# Autodesk Inventor assembly: Tattu 850mah 4S
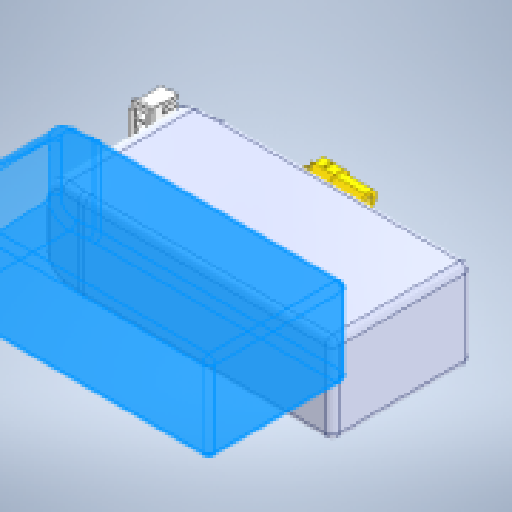
[picture p0: Inventor's stored thumbnail of the model, 512x512]
Saved by Autodesk Inventor 2023.2 (Build 272271000, 271)
## iProperties
Created: 2022-12-23
Part Number: Tattu 850mah 4S
Document SubType Name: Assembly
Designer: Nathan Cai
Mass: 57 g
Surface Area: 117.721 cm^2
Volume: 1.48579 cm^3
Density: 43.3194 g/cm^3
Author: Nathan Cai
## Documents named in this file (4)
- C:\Users\Nathan Cai\Documents\Inventor\Moon Cake V0.15\Tattu 4S 850mah\Tattu 850mah 4S.iam
- C:\Users\Nathan Cai\Documents\Inventor\Moon Cake V0.15\Tattu 4S 850mah\FUNDA 13.ipt
- C:\Users\Nathan Cai\Documents\Inventor\Moon Cake V0.15\Tattu 4S 850mah\JST XHP-4.ipt
- C:\Users\Nathan Cai\Documents\Inventor\Moon Cake V0.15\Tattu 4S 850mah\XdT30male.ipt
## Components (3 placed, 3 different names)
1. FUNDA 13:1 — Flush:2, Mate:2, Flush:3, Flush:4, Mate:3
2. JST XHP-4:1 — Flush:2, Mate:2, Flush:3
3. XdT30male:1 — Flush:4, Mate:3
## Relationships (5: Flush 3, Mate 2)
- Flush:2: FUNDA 13:1 ↔ JST XHP-4:1
- Mate:2: FUNDA 13:1 ↔ JST XHP-4:1
- Flush:3: FUNDA 13:1 ↔ JST XHP-4:1
- Flush:4: FUNDA 13:1 ↔ XdT30male:1
- Mate:3: FUNDA 13:1 ↔ XdT30male:1
